# Autodesk Inventor assembly: CIM Motor
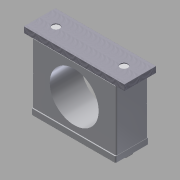
[picture p0: Inventor's stored thumbnail of the model, 180x180]
Saved by Autodesk Inventor 2013 (Build 170138000, 138)
## iProperties
Created: 2013-01-18
Part Number: CIM Motor
Document SubType Name: Assembly
Designer: Naphat
Author: Naphat
## Documents named in this file (5)
- C:\Users\Naphat\Google Drive\Robotics\FRC 2013\FRC2013 - LDU\Kiwi Robot\Imported Components\Motors\CIM Case\CIM Motor.iam
- C:\Users\Naphat\Google Drive\Robotics\FRC 2013\FRC2013 - LDU\Kiwi Robot\Imported Components\Motors\CIM Case\2.5 CIM mount.ipt
- C:\Users\Naphat\Google Drive\Robotics\FRC 2013\FRC2013 - LDU\Kiwi Robot\Imported Components\Motors\CIM Case\CIM Mount Top.ipt
- C:\Users\Naphat\Google Drive\Robotics\FRC 2013\FRC2013 - LDU\Kiwi Robot\Imported Components\Motors\CIM Case\CIM MountBase.ipt
- C:\Users\Naphat\Google Drive\Robotics\FRC 2013\FRC2013 - LDU\Kiwi Robot\Imported Components\Motors\CIM Case\CIM Mount Bolt.ipt
## Components (6 placed, 4 different names)
1. 2.5 CIM mount:1 — Mate:1, Mate:2, Mate:3, Mate:4, Mate:15, Mate:16, Mate:17
2. 2.5 CIM mount:2 — Mate:1, Mate:2, Mate:3, Mate:4, Mate:10, Mate:12, Mate:13, Mate:14
3. CIM Mount Top:1 — Mate:10, Mate:12, Mate:13, Mate:14, Mate:18, Mate:19, Mate:20, Mate:21
4. CIM MountBase:1 — Mate:15, Mate:16, Mate:17
5. CIM Mount Bolt:1 — Mate:18, Mate:19
6. CIM Mount Bolt:2 — Mate:20, Mate:21
## Relationships (15: Mate 15)
- Mate:1: 2.5 CIM mount:1 ↔ 2.5 CIM mount:2
- Mate:2: 2.5 CIM mount:1 ↔ 2.5 CIM mount:2
- Mate:3: 2.5 CIM mount:1 ↔ 2.5 CIM mount:2
- Mate:4: 2.5 CIM mount:1 ↔ 2.5 CIM mount:2
- Mate:10: 2.5 CIM mount:2 ↔ CIM Mount Top:1
- Mate:12: 2.5 CIM mount:2 ↔ CIM Mount Top:1
- Mate:13: 2.5 CIM mount:2 ↔ CIM Mount Top:1
- Mate:14: 2.5 CIM mount:2 ↔ CIM Mount Top:1
- Mate:15: 2.5 CIM mount:1 ↔ CIM MountBase:1
- Mate:16: 2.5 CIM mount:1 ↔ CIM MountBase:1
- Mate:17: 2.5 CIM mount:1 ↔ CIM MountBase:1
- Mate:18: CIM Mount Top:1 ↔ CIM Mount Bolt:1
- Mate:19: CIM Mount Top:1 ↔ CIM Mount Bolt:1
- Mate:20: CIM Mount Top:1 ↔ CIM Mount Bolt:2
- Mate:21: CIM Mount Top:1 ↔ CIM Mount Bolt:2
